# Autodesk Inventor assembly: ASY GBK 3210 central wall shield 4
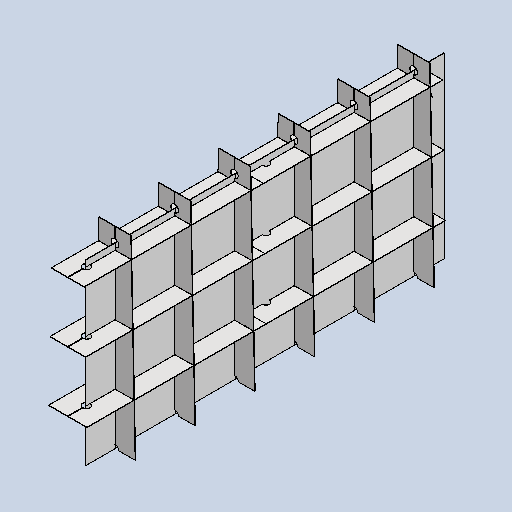
[picture p0: Inventor's stored thumbnail of the model, 512x512]
Saved by Autodesk Inventor 2026.2 (Build 302298010, 298A)
## iProperties
Created: 2026-05-19
Part Number: ASY GBK 3210 central wall shield 4
Document SubType Name: Assembly
Designer: pokla
Mass: 152628 g
Surface Area: 99280.6 cm^2
Volume: 19443.1 cm^3
Density: 7.85 g/cm^3
Author: admin
## Documents named in this file (7)
- C:\Users\admin\Documents\Inventor\GBK-Gubkinskiy\ASY GBK 3210 central wall shield 4.iam
- C:\Users\admin\Documents\Inventor\GBK-Gubkinskiy\GBK 3214 stringer 4.ipt
- C:\Users\admin\Documents\Inventor\GBK-Gubkinskiy\GBK 3215 stringer 5.ipt
- C:\Users\admin\Documents\Inventor\GBK-Gubkinskiy\GBK 3216 stringer 6.ipt
- C:\Users\admin\Documents\Inventor\GBK-Gubkinskiy\GBK 3214 shield 4.ipt
- C:\Users\admin\Documents\Inventor\GBK-Gubkinskiy\GBK 3212 central second rib.ipt
- C:\Users\admin\Documents\Inventor\GBK-Gubkinskiy\GBK 0101 main rib.ipt
## Components (25 placed, 5 different names)
1. GBK 3214 stringer 4.ipt:1 — Rigid:1, Rigid:10
2. GBK 3215 stringer 5.ipt:1 — Rigid:2, Rigid:11
3. GBK 3216 stringer 6.ipt:1 — Rigid:3, Rigid:12
4. GBK 3214 stringer 4.ipt:2 — Rigid:6, Rigid:7
5. GBK 3215 stringer 5.ipt:2 — Rigid:5, Rigid:8
6. GBK 3216 stringer 6.ipt:2 — Rigid:4, Rigid:9
7. GBK 3214 shield 4.ipt:1 — Mate:8, Mate:7, Flush:6, Mate:5, Flush:7, Flush:8, Mate:6
8. GBK 3214 stringer 4.ipt:3 — Rigid:7
9. GBK 3215 stringer 5.ipt:3 — Rigid:8
10. GBK 3216 stringer 6.ipt:3 — Rigid:9
11. GBK 3214 stringer 4.ipt:4 — Rigid:10
12. GBK 3215 stringer 5.ipt:4 — Rigid:11
13. GBK 3216 stringer 6.ipt:4 — Rigid:12
14. GBK 3212 central second rib.ipt:1 — Mate:5, Flush:4, Rigid:6, Rigid:5, Rigid:4, Mate:5, Flush:7, Flush:8
15. GBK 3212 central second rib.ipt:2 — Mate:6, Flush:4, Rigid:1, Rigid:2, Rigid:3, Mate:6
16. GBK 3212 central second rib.ipt:3
17. GBK 3212 central second rib.ipt:4
18. GBK 3212 central second rib.ipt:5
19. GBK 3212 central second rib.ipt:6
20. GBK 3212 central second rib.ipt:7
21. GBK 3212 central second rib.ipt:8
22. GBK 3212 central second rib.ipt:9
23. GBK 3212 central second rib.ipt:10
24. GBK 3212 central second rib.ipt:11
25. GBK 3212 central second rib.ipt:12
## Component patterns: (6 elements, first: GBK 3212 central second rib.ipt:1 + GBK 3212 central second rib.ipt:2)
## Relationships (22: WeldJoint 12, Mate 6, Flush 4)
- Mate:6: GBK 3212 central second rib.ipt:2
- Mate:5: GBK 3212 central second rib.ipt:1
- Flush:4: GBK 3212 central second rib.ipt:1 ↔ GBK 3212 central second rib.ipt:2
- Mate:8: GBK 3214 shield 4.ipt:1
- Mate:7: GBK 3214 shield 4.ipt:1
- Rigid:1 [WeldJoint] (4 mm): GBK 3214 stringer 4.ipt:1 ↔ GBK 3212 central second rib.ipt:2
- Rigid:2 [WeldJoint] (4 mm): GBK 3215 stringer 5.ipt:1 ↔ GBK 3212 central second rib.ipt:2
- Rigid:3 [WeldJoint] (4 mm): GBK 3216 stringer 6.ipt:1 ↔ GBK 3212 central second rib.ipt:2
- Rigid:6 [WeldJoint] (4 mm): GBK 3214 stringer 4.ipt:2 ↔ GBK 3212 central second rib.ipt:1
- Rigid:5 [WeldJoint] (4 mm): GBK 3215 stringer 5.ipt:2 ↔ GBK 3212 central second rib.ipt:1
- Rigid:4 [WeldJoint] (4 mm): GBK 3216 stringer 6.ipt:2 ↔ GBK 3212 central second rib.ipt:1
- Flush:6: GBK 3214 shield 4.ipt:1
- Mate:5: GBK 3214 shield 4.ipt:1 ↔ GBK 3212 central second rib.ipt:1
- Flush:7: GBK 3214 shield 4.ipt:1 ↔ GBK 3212 central second rib.ipt:1
- Flush:8 (250 mm): GBK 3214 shield 4.ipt:1 ↔ GBK 3212 central second rib.ipt:1
- Rigid:7 [WeldJoint]: GBK 3214 stringer 4.ipt:2 ↔ GBK 3214 stringer 4.ipt:3
- Rigid:8 [WeldJoint]: GBK 3215 stringer 5.ipt:2 ↔ GBK 3215 stringer 5.ipt:3
- Rigid:9 [WeldJoint]: GBK 3216 stringer 6.ipt:2 ↔ GBK 3216 stringer 6.ipt:3
- Rigid:10 [WeldJoint]: GBK 3214 stringer 4.ipt:1 ↔ GBK 3214 stringer 4.ipt:4
- Rigid:11 [WeldJoint]: GBK 3215 stringer 5.ipt:1 ↔ GBK 3215 stringer 5.ipt:4
- Rigid:12 [WeldJoint]: GBK 3216 stringer 6.ipt:1 ↔ GBK 3216 stringer 6.ipt:4
- Mate:6: GBK 3214 shield 4.ipt:1 ↔ GBK 3212 central second rib.ipt:2
## Named parameters: Шаг_шпангоутов = 496.66667 mm
